# Autodesk Inventor assembly: DriveBase Assembly
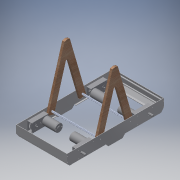
[picture p0: Inventor's stored thumbnail of the model, 180x180]
Saved by Autodesk Inventor 2017 (Build 210142000, 142)
## iProperties
Created: 2017-04-25
Part Number: DriveBase Assembly
Document SubType Name: Assembly
Designer: admin
Author: admin
## Documents named in this file (6)
- C:\Users\admin\Desktop\RoboEaglesCad2018\DriveBase Assembly.iam
- C:\Users\admin\Desktop\RoboEaglesCad2018\DriveBaseSidePanel.ipt
- C:\Users\admin\Desktop\RoboEaglesCad2018\DriveBaseFront.ipt
- C:\Users\admin\Desktop\RoboEaglesCad2018\Toughbox+Nano+All+Shafts+v2(ForUseInModel).iam
- C:\Users\admin\Desktop\RoboEaglesCad2018\InsideChurroBodySupport.ipt
- C:\Users\admin\Desktop\RoboEaglesCad2018\aFrameBase.ipt
## Components (12 placed, 5 different names)
1. DriveBaseSidePanel:1 — Flush:1, Flush:2, Mate:3, Mate:4, Mate:5, Mate:6, Flush:4, Flush:5, Mate:12, Mate:13, Insert:3, Insert:4, Angle:1, Angle:2, Mate:15
2. DriveBaseFront:1 — Flush:1, Flush:2, Mate:1, Mate:2, Mate:3, Mate:4, Mate:7, Mate:10
3. DriveBaseSidePanel:2 — Mate:1, Mate:2, Flush:3, Flush:6, Flush:7, Mate:11, Mate:14, Insert:1, Insert:2, Flush:8, Flush:9
4. DriveBaseFront:2 — Mate:5, Mate:6, Flush:3, Mate:8, Mate:9
5. Toughbox+Nano+All+Shafts+v2(ForUseInModel):1 [sub-assembly] — Flush:5, Mate:7, Mate:12
6. Toughbox+Nano+All+Shafts+v2(ForUseInModel):2 [sub-assembly] — Flush:4, Mate:8, Mate:13
7. Toughbox+Nano+All+Shafts+v2(ForUseInModel):3 [sub-assembly] — Flush:6, Mate:10, Mate:11
8. Toughbox+Nano+All+Shafts+v2(ForUseInModel):4 [sub-assembly] — Flush:7, Mate:9, Mate:14
9. InsideChurroBodySupport:1 — Insert:2, Insert:3, Angle:1, Mate:16
10. InsideChurroBodySupport:2 — Insert:1, Insert:4, Angle:2, Mate:17
11. aFrameBase:1 — Flush:8, Flush:9
12. aFrameBase:2 — Mate:15, Mate:16, Mate:17
## Relationships (32: Mate 17, Flush 9, Insert 4, Angle 2)
- Flush:1: DriveBaseSidePanel:1 ↔ DriveBaseFront:1
- Flush:2: DriveBaseSidePanel:1 ↔ DriveBaseFront:1
- Mate:1: DriveBaseFront:1 ↔ DriveBaseSidePanel:2
- Mate:2: DriveBaseFront:1 ↔ DriveBaseSidePanel:2
- Mate:3: DriveBaseSidePanel:1 ↔ DriveBaseFront:1
- Mate:4: DriveBaseSidePanel:1 ↔ DriveBaseFront:1
- Mate:5: DriveBaseSidePanel:1 ↔ DriveBaseFront:2
- Mate:6: DriveBaseSidePanel:1 ↔ DriveBaseFront:2
- Flush:3: DriveBaseSidePanel:2 ↔ DriveBaseFront:2
- Flush:4 (12.7 mm): DriveBaseSidePanel:1 ↔ Toughbox+Nano+All+Shafts+v2(ForUseInModel):2
- Flush:5 (12.7 mm): DriveBaseSidePanel:1 ↔ Toughbox+Nano+All+Shafts+v2(ForUseInModel):1
- Flush:6 (12.7 mm): DriveBaseSidePanel:2 ↔ Toughbox+Nano+All+Shafts+v2(ForUseInModel):3
- Flush:7 (12.7 mm): DriveBaseSidePanel:2 ↔ Toughbox+Nano+All+Shafts+v2(ForUseInModel):4
- Mate:7 (85.725 mm): DriveBaseFront:1 ↔ Toughbox+Nano+All+Shafts+v2(ForUseInModel):1
- Mate:8 (85.725 mm): DriveBaseFront:2 ↔ Toughbox+Nano+All+Shafts+v2(ForUseInModel):2
- Mate:9 (85.725 mm): DriveBaseFront:2 ↔ Toughbox+Nano+All+Shafts+v2(ForUseInModel):4
- Mate:10 (85.725 mm): DriveBaseFront:1 ↔ Toughbox+Nano+All+Shafts+v2(ForUseInModel):3
- Mate:11: DriveBaseSidePanel:2 ↔ Toughbox+Nano+All+Shafts+v2(ForUseInModel):3
- Mate:12: DriveBaseSidePanel:1 ↔ Toughbox+Nano+All+Shafts+v2(ForUseInModel):1
- Mate:13: DriveBaseSidePanel:1 ↔ Toughbox+Nano+All+Shafts+v2(ForUseInModel):2
- Mate:14: DriveBaseSidePanel:2 ↔ Toughbox+Nano+All+Shafts+v2(ForUseInModel):4
- Insert:1: DriveBaseSidePanel:2 ↔ InsideChurroBodySupport:2
- Insert:2: DriveBaseSidePanel:2 ↔ InsideChurroBodySupport:1
- Insert:3: DriveBaseSidePanel:1 ↔ InsideChurroBodySupport:1
- Insert:4: DriveBaseSidePanel:1 ↔ InsideChurroBodySupport:2
- Angle:1 (0 deg): DriveBaseSidePanel:1 ↔ InsideChurroBodySupport:1
- Angle:2 (0 deg): DriveBaseSidePanel:1 ↔ InsideChurroBodySupport:2
- Flush:8: DriveBaseSidePanel:2 ↔ aFrameBase:1
- Flush:9: DriveBaseSidePanel:2 ↔ aFrameBase:1
- Mate:15: DriveBaseSidePanel:1 ↔ aFrameBase:2
- Mate:16: InsideChurroBodySupport:1 ↔ aFrameBase:2
- Mate:17: InsideChurroBodySupport:2 ↔ aFrameBase:2
